# Autodesk Inventor assembly: Minimo
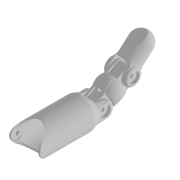
[picture p0: Inventor's stored thumbnail of the model, 180x180]
Saved by Autodesk Inventor 2020 (Build 240168000, 168)
## iProperties
Created: 2021-03-24
Part Number: Minimo
Document SubType Name: Assembly
Designer: deox
Author: deox
## Documents named in this file (7)
- C:\Users\deox\Desktop\TCC\Inventor Files\Dedo Kick\Minimo.iam
- C:\Users\deox\Desktop\TCC\Inventor Files\Dedo Kick\Socket_Minimo.ipt
- C:\Users\deox\Desktop\TCC\Inventor Files\Dedo Kick\Base_Minimo.ipt
- C:\Users\deox\Desktop\TCC\Inventor Files\Dedo Kick\Middle_Minimo.ipt
- C:\Users\deox\Desktop\TCC\Inventor Files\Dedo Kick\ShameHider_Minimo.ipt
- C:\Users\deox\Desktop\TCC\Inventor Files\Dedo Kick\Tip_Minimo_ScaledDown.ipt
- C:\Users\deox\Desktop\TCC\Inventor Files\Dedo Kick\TipTip_Minimo.ipt
## Components (6 placed, 6 different names)
1. Socket_Minimo:1 — Mate:12, Mate:13, Angle:2
2. Base_Minimo:1 — Mate:12, Mate:13, Angle:2, Mate:14, Mate:15
3. Middle_Minimo:1 — Mate:14, Mate:15, Mate:16, Mate:17, Mate:18, Mate:19, Mate:20
4. ShameHider_Minimo:1 — Mate:16, Mate:17, Mate:18
5. Tip_Minimo_ScaledDown:1 — Mate:19, Mate:20, Mate:21
6. TipTip_Minimo:1 — Mate:21
## Relationships (11: Mate 10, Angle 1)
- Mate:12: Socket_Minimo:1 ↔ Base_Minimo:1
- Mate:13: Socket_Minimo:1 ↔ Base_Minimo:1
- Angle:2 (0 deg): Socket_Minimo:1 ↔ Base_Minimo:1
- Mate:14: Base_Minimo:1 ↔ Middle_Minimo:1
- Mate:15: Base_Minimo:1 ↔ Middle_Minimo:1
- Mate:16: Middle_Minimo:1 ↔ ShameHider_Minimo:1
- Mate:17: Middle_Minimo:1 ↔ ShameHider_Minimo:1
- Mate:18: Middle_Minimo:1 ↔ ShameHider_Minimo:1
- Mate:19: Middle_Minimo:1 ↔ Tip_Minimo_ScaledDown:1
- Mate:20: Middle_Minimo:1 ↔ Tip_Minimo_ScaledDown:1
- Mate:21: Tip_Minimo_ScaledDown:1 ↔ TipTip_Minimo:1
